# Autodesk Inventor assembly: FA[23]
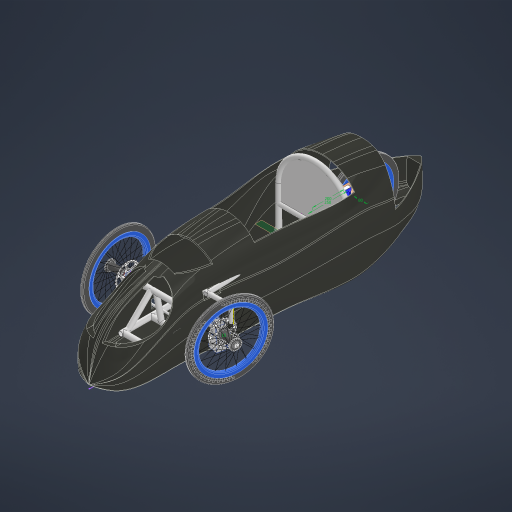
[picture p0: Inventor's stored thumbnail of the model, 512x512]
Saved by Autodesk Inventor 2024 (Build 280153000, 153)
## iProperties
Created: 2023-01-27
Part Number: FA[23]
Document SubType Name: Assembly
Designer: juanj
Author: juanj
## Documents named in this file (22)
- C:\Users\juanj\Documents\Documentos\Unisabana\Shell\C23 DESING\A23[F]\FA[23].iam
- C:\Users\juanj\Documents\Documentos\Unisabana\Shell\C23 DESING\A23[F]\PFA23[F]\FB23[F].ipt
- C:\Users\juanj\Documents\Documentos\Unisabana\Shell\C23 DESING\A23[F]\PFA23[F]\TW23[F].ipt
- C:\Users\juanj\Documents\Documentos\Unisabana\Shell\C23 DESING\A23[F]\PFA23[F]\W23[F].ipt
- C:\Users\juanj\Documents\Documentos\Unisabana\Shell\C23 DESING\A23[F]\PFA23[F]\BU23[F].ipt
- C:\Users\juanj\Documents\Documentos\Unisabana\Shell\C23 DESING\A23[F]\PFA23[F]\C23[F].ipt
- C:\Users\juanj\Documents\Documentos\Unisabana\Shell\C23 DESING\A23[F]\PFA23[F]\R23[F].ipt
- C:\Users\juanj\Documents\Documentos\Unisabana\Shell\C23 DESING\A23[F]\PFA23[F]\S23[F].ipt
- C:\Users\juanj\Documents\Documentos\Unisabana\Shell\C23 DESING\A23[F]\PFA23[F]\N23[1][F].ipt
- C:\Users\juanj\Documents\Documentos\Unisabana\Shell\C23 DESING\A23[F]\PFA23[F]\N23[F][2].ipt
- C:\Users\juanj\Documents\Documentos\Unisabana\Shell\C23 DESING\A23[F]\PFA23[F]\D23[F].iam
- C:\Users\juanj\Documents\Documentos\Unisabana\Shell\C23 DESING\A23[F]\PFA23[F]\SW23[F].ipt
- C:\Users\juanj\Documents\Documentos\Unisabana\Shell\C23 DESING\A23[F]\PFA23[F]\M23[F].ipt
- C:\Users\juanj\Documents\Documentos\Unisabana\Shell\C23 DESING\A23[F]\PFA23[F]\ET23[F].iam
- C:\Users\juanj\Documents\Documentos\Unisabana\Shell\C23 DESING\A23[F]\PFA23[F]\BW23[F].ipt
- C:\Users\juanj\Documents\Documentos\Unisabana\Shell\C23 DESING\A23[F]\PFA23[F]\HB[F].ipt
- C:\Users\juanj\Documents\Documentos\Unisabana\Shell\C23 DESING\A23[F]\PFA23[F]\B23[F]_MIR2.ipt
- C:\Users\juanj\Documents\Documentos\Unisabana\Shell\C23 DESING\A23[F]\PFA23[F]\B23[F1].ipt
- C:\Users\juanj\Documents\Documentos\Unisabana\Shell\C23[1stD]\C23[L][FD1].ipt
- C:\Users\juanj\Documents\Documentos\Unisabana\Shell\C23[1stD]\C23[R][FD1].ipt
- C:\Users\juanj\Documents\Documentos\Unisabana\Shell\C23[1stD]\DC23[L][FD1].ipt
- C:\Users\juanj\Documents\Documentos\Unisabana\Shell\C23[1stD]\DC23[R][FD1].ipt
## Components (30 placed, 21 different names)
1. TW23[F]:1 — Insertar:4
2. BU23[F]:1 — Insertar:14, Insertar:21, Insert:53
3. C23[F]:1 — Insertar:3
4. R23[F]:3 — Insertar:7, Insert:43
5. R23[F]:4 — Insertar:8
6. N23[F][2]:1 — Insertar:21
7. N23[1][F]:1 — Insert:45
8. S23[F]:2 — Insert:47
9. S23[F]:1 — Insert:44
10. D23[F]:1 [sub-assembly] — Insert:49, Mate:4
11. SW23[F]:1
12. M23[F]:1 — Insertar:37
13. ET23[F]:1 [sub-assembly] — Coincidencia:2, Coincidencia:3, Nivelación:6
14. BW23[F]:1 — Insertar:38, Ángulo:8
15. B23[F]_MIR2:1 — Insert:39, Angle:10, Insert:50, Angle:13
16. HB[F]:2 — Insert:40, Angle:9
17. B23[F1]:1 — Insert:40, Angle:9, Insert:51, Angle:14
18. FB23[F]:1 — Insertar:3, Insertar:4, Insertar:5, Insertar:6, Insertar:7, Insertar:8, Insertar:37, Nivelación:3, Nivelación:4, Insertar:38, Ángulo:8, Nivelación:5
19. W23[F]:1 — Insertar:14
20. BU23[F]:2 — Insertar:15, Insertar:20, Insert:52
21. R23[F]:1 — Insertar:5, Insert:46
22. N23[1][F]:2 — Insert:48
23. HB[F]:3 — Insert:39, Angle:10
24. N23[F][2]:2 — Insertar:20
25. W23[F]:2 — Insertar:15
26. R23[F]:2 — Insertar:6
27. C23[L][FD1]:1 — Insert:41, Angle:11, Insert:46, Insert:47, Insert:51, Insert:52
28. C23[R][FD1]:1 — Insert:42, Angle:12, Insert:43, Insert:44, Insert:50, Insert:53
29. DC23[L][FD1]:1 — Insert:41, Angle:11, Insert:48, Insert:49, Angle:14
30. DC23[R][FD1]:1 — Insert:42, Angle:12, Insert:45, Mate:4, Angle:13
## Relationships (41: Insert 27, Angle 7, Flush 4, Mate 3)
- Insertar:3: C23[F]:1 ↔ FB23[F]:1
- Insertar:4: TW23[F]:1 ↔ FB23[F]:1
- Insertar:5: FB23[F]:1 ↔ R23[F]:1
- Insertar:6: FB23[F]:1 ↔ R23[F]:2
- Insertar:7: R23[F]:3 ↔ FB23[F]:1
- Insertar:8: R23[F]:4 ↔ FB23[F]:1
- Insertar:14: BU23[F]:1 ↔ W23[F]:1
- Insertar:15: BU23[F]:2 ↔ W23[F]:2
- Insertar:20: BU23[F]:2 ↔ N23[F][2]:2
- Insertar:21: BU23[F]:1 ↔ N23[F][2]:1
- Insertar:37: M23[F]:1 ↔ FB23[F]:1
- Nivelación:3 [Flush] (30 mm): FB23[F]:1
- Nivelación:4 [Flush] (29 mm): FB23[F]:1
- Coincidencia:2 [Mate]: ET23[F]:1
- Coincidencia:3 [Mate]: ET23[F]:1
- Insertar:38 (106.5 mm): BW23[F]:1 ↔ FB23[F]:1
- Ángulo:8 [Angle] (180 deg): BW23[F]:1 ↔ FB23[F]:1
- Nivelación:5 [Flush] (-50 mm): FB23[F]:1
- Nivelación:6 [Flush]: ET23[F]:1
- Insert:39: B23[F]_MIR2:1 ↔ HB[F]:3
- Insert:40: HB[F]:2 ↔ B23[F1]:1
- Angle:9 (0 deg): HB[F]:2 ↔ B23[F1]:1
- Angle:10 (0 deg): B23[F]_MIR2:1 ↔ HB[F]:3
- Insert:41: C23[L][FD1]:1 ↔ DC23[L][FD1]:1
- Angle:11 (0 deg): C23[L][FD1]:1 ↔ DC23[L][FD1]:1
- Insert:42: C23[R][FD1]:1 ↔ DC23[R][FD1]:1
- Angle:12 (0 deg): C23[R][FD1]:1 ↔ DC23[R][FD1]:1
- Insert:43: R23[F]:3 ↔ C23[R][FD1]:1
- Insert:44: S23[F]:1 ↔ C23[R][FD1]:1
- Insert:45: N23[1][F]:1 ↔ DC23[R][FD1]:1
- Insert:46: R23[F]:1 ↔ C23[L][FD1]:1
- Insert:47: S23[F]:2 ↔ C23[L][FD1]:1
- Insert:48: N23[1][F]:2 ↔ DC23[L][FD1]:1
- Insert:49: D23[F]:1 ↔ DC23[L][FD1]:1
- Mate:4: D23[F]:1 ↔ DC23[R][FD1]:1
- Insert:50: B23[F]_MIR2:1 ↔ C23[R][FD1]:1
- Angle:13 (0 deg): B23[F]_MIR2:1 ↔ DC23[R][FD1]:1
- Insert:51: B23[F1]:1 ↔ C23[L][FD1]:1
- Angle:14 (0 deg): B23[F1]:1 ↔ DC23[L][FD1]:1
- Insert:52: BU23[F]:2 ↔ C23[L][FD1]:1
- Insert:53: BU23[F]:1 ↔ C23[R][FD1]:1
